# Autodesk Inventor assembly: HCMUTE-CDT23-PLXR_ASEMBLY
(part 2 of 2)
- Mate:182: HCMUTE-CDT23-MOTOR_DC24V-100RPM-XD42GA775:1 ↔ HCMUTE-CDT23-GA_DC:1
- Mate:183: HCMUTE-CDT23-MOTOR_DC24V-100RPM-XD42GA775:1 ↔ HCMUTE-CDT23-PULLY_S5M-15X15X8:1
- Mate:184 (5 mm): HCMUTE-CDT23-PULLY_S5M-15X15X8:1 ↔ HCMUTE-CDT23-GA_DC:1
- Mate:185: HCMUTE-CDT23-FRAME_ASEMBLY:1 ↔ HCMUTE-CDT23-GA_DC:1
- Mate:186 (59.9799 mm): HCMUTE-CDT23-FRAME_ASEMBLY:1 ↔ HCMUTE-CDT23-GA_DC:1
- Flush:25: HCMUTE-CDT23-PULLY_S5M-30X15X12:2 ↔ HCMUTE-CDT23-PULLY_S5M-15X15X8:1
- Mate:187: HCMUTE-CDT23-PULLY_S5M-15X15X8:1 ↔ 2309HCMUTE-CDT23-BELT_S5M-355X71X15:1
- Mate:188 (1 mm): HCMUTE-CDT23-PULLY_S5M-15X15X8:1 ↔ 2309HCMUTE-CDT23-BELT_S5M-355X71X15:1
- Mate:189: HCMUTE-CDT23-TRUC_DAN:1 ↔ 2309HCMUTE-CDT23-BELT_S5M-355X71X15:1
- Mate:190: HCMUTE-CDT23-FRAME_ASEMBLY:1 ↔ HCMUTE-CDT23-BAT_TRUC_DAN:2
- Mate:191: HCMUTE-CDT23-BAT_TRUC_DAN:2 ↔ HCMUTE-CDT23-GOI_DO_KFL003:2
- Mate:192: HCMUTE-CDT23-BAT_TRUC_DAN:2 ↔ ISO 4762 M6 x 25:3
- Mate:193: HCMUTE-CDT23-BAT_TRUC_DAN:2 ↔ ISO 4762 M6 x 25:4
- Mate:194: HCMUTE-CDT23-BAT_TRUC_DAN:1 ↔ ISO 4762 M6 x 12:1
- Mate:196: HCMUTE-CDT23-BAT_TRUC_DAN:1 ↔ ISO 4762 M6 x 12:2
- Mate:199: HCMUTE-CDT23-OP_GA-STEP-42:1 ↔ HCMUTE-CDT23-OP_NDH-2020X500:1
- Flush:26 (-9.75 mm): HCMUTE-CDT23-OP_GA-STEP-42:1 ↔ HCMUTE-CDT23-OP_NDH-2020X500:1
- Flush:27 (-40 mm): HCMUTE-CDT23-OP_GA-STEP-42:1 ↔ HCMUTE-CDT23-OP_NDH-2020X500:1
- Mate:200: HCMUTE-CDT23-OP_GA-STEP-42:1 ↔ HCMUTE-CDT23-OP_STEP-42:1
- Mate:201: HCMUTE-CDT23-OP_GA-STEP-42:1 ↔ HCMUTE-CDT23-OP_STEP-42:1
- Mate:202: HCMUTE-CDT23-OP_GA-CONLAN:1 ↔ HCMUTE-CDT23-OP_NDH-2020X500:1
- Flush:28 (-30 mm): HCMUTE-CDT23-OP_GA-CONLAN:1 ↔ HCMUTE-CDT23-OP_NDH-2020X500:1
- Mate:203 (3 mm): HCMUTE-CDT23-BTC_ASEMBLY:1 ↔ HCMUTE-CDT23-OP_NDH-2020X500:1
- Mate:206: HCMUTE-CDT23-FRAME_ASEMBLY:1 ↔ HCMUTE-CDT23-OP_TAMLOT:1
- Flush:30: HCMUTE-CDT23-FRAME_ASEMBLY:1 ↔ HCMUTE-CDT23-OP_TAMLOT:1
- Flush:31: HCMUTE-CDT23-OP_NDH-2020X500:1 ↔ HCMUTE-CDT23-OP_TAMLOT:1
- Mate:207: 301818 302828.1:1 ↔ HCMUTE-CDT23-OP_TAMLOT:1
- Mate:208: HCMUTE-CDT23-OP_NDH-2020X500:1 ↔ 301818 302828.1:1
- Flush:32 (6 mm): HCMUTE-CDT23-FRAME_ASEMBLY:1 ↔ 301818 302828.1:1
- Mate:209: HCMUTE-CDT23-OP_TAMLOT:1 ↔ 301818 302828.1:2
- Mate:210: HCMUTE-CDT23-OP_NDH-2020X500:1 ↔ 301818 302828.1:2
- Flush:33: 301818 302828.1:1 ↔ 301818 302828.1:2
- Mate:211: HCMUTE-CDT23-OP_TAMLOT:1 ↔ ISO 4762 M5 x 12:1
- Mate:212: 301818 302828.1:2 ↔ ISO 4762 M5 x 12:1
- Mate:213: HCMUTE-CDT23-OP_TAMLOT:1 ↔ ISO 4762 M5 x 12:2
- Mate:214: 301818 302828.1:1 ↔ ISO 4762 M5 x 12:2
- Flush:34 (-9.75 mm): HCMUTE-CDT23-OP_GA-CONLAN:1 ↔ HCMUTE-CDT23-OP_NDH-2020X500:1
- Flush:35 (-20 mm): HCMUTE-CDT23-FRAME_ASEMBLY:1 ↔ HCMUTE-CDT23-OP_NDH-2020X500:1
- Mate:215: HCMUTE-CDT23-OP_STEP-42:1 ↔ HCMUTE-CDT23-OP_PULLY-GT2-30X6X5:1
- Mate:216 (7 mm): HCMUTE-CDT23-OP_GA-STEP-42:1 ↔ HCMUTE-CDT23-OP_PULLY-GT2-30X6X5:1
- Mate:217: HCMUTE-CDT23-OP_GA-STEP-42:1 ↔ ISO 4762 M5 x 8:1
- Mate:218: HCMUTE-CDT23-OP_GA-STEP-42:1 ↔ ISO 4762 M5 x 8:1
- Mate:219: HCMUTE-CDT23-OP_GA-STEP-42:1 ↔ ISO 4762 M5 x 8:2
- Mate:220: HCMUTE-CDT23-OP_GA-STEP-42:1 ↔ ISO 4762 M5 x 8:2
- Mate:221: HCMUTE-CDT23-OP_GA-CONLAN:1 ↔ ISO 4762 M5 x 8:3
- Mate:222: HCMUTE-CDT23-OP_GA-CONLAN:1 ↔ ISO 4762 M5 x 8:3
- Mate:223: HCMUTE-CDT23-OP_GA-CONLAN:1 ↔ ISO 4762 M5 x 8:4
- Mate:224: HCMUTE-CDT23-OP_GA-CONLAN:1 ↔ ISO 4762 M5 x 8:4
- Mate:225: HCMUTE-CDT23-OP_GA-CONLAN:1 ↔ HCMUTE-CDT23-OP_RONG-ROC:1
- Mate:226: HCMUTE-CDT23-OP_GA-CONLAN:1 ↔ HCMUTE-CDT23-OP_RONG-ROC:1
- Mate:227: HCMUTE-CDT23-OP_V-WHEEL:1 ↔ HCMUTE-CDT23-OP_BASE-PLATE:1
- Mate:228: HCMUTE-CDT23-OP_V-WHEEL:1 ↔ HCMUTE-CDT23-OP_BASE-PLATE:1
- Mate:229: HCMUTE-CDT23-OP_BASE-PLATE:1 ↔ HCMUTE-CDT23-OP_V-WHEEL:3
- Mate:230: HCMUTE-CDT23-OP_BASE-PLATE:1 ↔ HCMUTE-CDT23-OP_V-WHEEL:3
- Mate:231: HCMUTE-CDT23-OP_BASE-PLATE:1 ↔ HCMUTE-CDT23-OP_V-WHEEL:4
- Mate:232: HCMUTE-CDT23-OP_BASE-PLATE:1 ↔ HCMUTE-CDT23-OP_V-WHEEL:4
- Mate:233: HCMUTE-CDT23-OP_BASE-PLATE:1 ↔ HCMUTE-CDT23-OP_V-WHEEL:5
- Mate:234: HCMUTE-CDT23-OP_BASE-PLATE:1 ↔ HCMUTE-CDT23-OP_V-WHEEL:5
- Angle:3 (0 deg): HCMUTE-CDT23-OP_BASE-PLATE:1
- Flush:37: HCMUTE-CDT23-OP_V-WHEEL:1
- Flush:38: HCMUTE-CDT23-OP_V-WHEEL:1
- Symmetry:1
- Flush:39: HCMUTE-CDT23-OP_NDH-2020X500:1
- Flush:40: HCMUTE-CDT23-OP_NDH-2020X500:1
- Symmetry:2
- Mate:235
- Mate:236: HCMUTE-CDT23-OP_GA-CONLAN:1 ↔ HCMUTE-CDT23-OP_BASE-PLATE:1
- Mate:273: HCMUTE-CDT23-OP_DVCAM:1 ↔ Assembly_HCMUTE-CDT23-CAMERA_C270Logitech c270 Assembly:1
- Mate:274: HCMUTE-CDT23-OP_DVCAM:1 ↔ Assembly_HCMUTE-CDT23-CAMERA_C270Logitech c270 Assembly:1
- Mate:275: HCMUTE-CDT23-OP_DVCAM:1 ↔ Assembly_HCMUTE-CDT23-CAMERA_C270Logitech c270 Assembly:1
- Mate:276: HCMUTE-CDT23-FRAME_ASEMBLY:1 ↔ HCMUTE-CDT23-KXL_CHAN-GA:1
- Flush:52 (-15 mm): HCMUTE-CDT23-FRAME_ASEMBLY:1 ↔ HCMUTE-CDT23-KXL_CHAN-GA:1
- Mate:277: HCMUTE-CDT23-FRAME_ASEMBLY:1 ↔ HCMUTE-CDT23-KXL_CHAN-GA:1
- Mate:278: HCMUTE-CDT23-KXL_CHAN-GA:1 ↔ ISO 4762 M6 x 10:10
- Mate:279: HCMUTE-CDT23-KXL_CHAN-GA:1 ↔ ISO 4762 M6 x 10:10
- Mate:280: HCMUTE-CDT23-KXL_CHAN-GA:1 ↔ ISO 4762 M6 x 10:9
- Mate:281: HCMUTE-CDT23-KXL_CHAN-GA:1 ↔ ISO 4762 M6 x 10:9
- Mate:282: HCMUTE-CDT23-FRAME_ASEMBLY:1 ↔ HCMUTE-CDT23-KXL_CHAN-GA:2
- Mate:283: HCMUTE-CDT23-FRAME_ASEMBLY:1 ↔ HCMUTE-CDT23-KXL_CHAN-GA:2
- Flush:53: HCMUTE-CDT23-KXL_CHAN-GA:1 ↔ HCMUTE-CDT23-KXL_CHAN-GA:2
- Mate:284 (6 mm): HCMUTE-CDT23-FRAME_ASEMBLY:1 ↔ HCMUTE-CDT23-KXL_CHAN-GA:3
- Mate:285: HCMUTE-CDT23-FRAME_ASEMBLY:1 ↔ HCMUTE-CDT23-KXL_CHAN-GA:3
- Flush:54: HCMUTE-CDT23-KXL_CHAN-GA:2 ↔ HCMUTE-CDT23-KXL_CHAN-GA:3
- Mate:286: HCMUTE-CDT23-KXL_CHAN-GA:1 ↔ HCMUTE-CDT23-KXL_A01:1
- Mate:287: HCMUTE-CDT23-KXL_CHAN-GA:1 ↔ HCMUTE-CDT23-KXL_A01:1
- Mate:288: HCMUTE-CDT23-KXL_A01:1 ↔ 2309HCMUTE-CDT23-KXL_GA-VUONG:1
- Flush:55: HCMUTE-CDT23-KXL_A01:1 ↔ 2309HCMUTE-CDT23-KXL_GA-VUONG:1
- Mate:289: HCMUTE-CDT23-KXL_A01:1 ↔ 2309HCMUTE-CDT23-KXL_GA-VUONG:1
- Mate:290: HCMUTE-CDT23-KXL_A01:1 ↔ 2309HCMUTE-CDT23-KXL_GA-VUONG:2
- Flush:56: 2309HCMUTE-CDT23-KXL_GA-VUONG:1 ↔ 2309HCMUTE-CDT23-KXL_GA-VUONG:2
- Mate:291: HCMUTE-CDT23-KXL_A01:1 ↔ 2309HCMUTE-CDT23-KXL_GA-VUONG:2
- Mate:292: HCMUTE-CDT23-KXL_A01:1 ↔ 2309HCMUTE-CDT23-KXL_GA-VUONG:3
- Mate:293: HCMUTE-CDT23-KXL_A01:1 ↔ 2309HCMUTE-CDT23-KXL_GA-VUONG:3
- Flush:57: HCMUTE-CDT23-KXL_A01:1 ↔ 2309HCMUTE-CDT23-KXL_GA-VUONG:3
- Mate:296: HCMUTE-CDT23-KXL_CHAN-GA:3 ↔ ISO 4032 M5:1
- Mate:309: 2309HCMUTE-CDT23-KXL_GA-VUONG:4 ↔ ISO 4032 M5:5
- Mate:310: ISO 4032 M5:5 ↔ ISO 4762 M5 x 12:8
- Mate:311: ISO 4032 M5:4 ↔ ISO 4762 M5 x 12:9
- Mate:312: ISO 4032 M5:4 ↔ 2309HCMUTE-CDT23-KXL_GA-VUONG:7
- Mate:313: HCMUTE-CDT23-KXL_A01:1 ↔ HCMUTE-CDT23-KXL_A03:1
- Mate:315: ISO 4762 M5 x 12:14 ↔ 2309HCMUTE-CDT23-KXL_GA-VUONG:7
- Mate:316: HCMUTE-CDT23-KXL_A03:1 ↔ ISO 4762 M5 x 12:14
- Mate:317: ISO 4032 M5:10 ↔ 2309HCMUTE-CDT23-KXL_GA-VUONG:7
- Mate:318: ISO 4032 M5:10 ↔ ISO 4762 M5 x 12:14
- Mate:319: HCMUTE-CDT23-KXL_A03:1 ↔ HCMUTE-CDT23-KXL_A02:2
- Flush:61: HCMUTE-CDT23-KXL_A03:1 ↔ HCMUTE-CDT23-KXL_A02:2
- Flush:62 (3 mm): HCMUTE-CDT23-KXL_A03:1 ↔ HCMUTE-CDT23-KXL_A02:2
- Mate:320: HCMUTE-CDT23-FRAME_ASEMBLY:1 ↔ HCMUTE-CDT23-KXL_CHAN-GA:4
- Flush:63 (-16 mm): HCMUTE-CDT23-FRAME_ASEMBLY:1 ↔ HCMUTE-CDT23-KXL_CHAN-GA:4
- Mate:321: HCMUTE-CDT23-FRAME_ASEMBLY:1 ↔ HCMUTE-CDT23-KXL_CHAN-GA:4
- Mate:322: HCMUTE-CDT23-FRAME_ASEMBLY:1 ↔ HCMUTE-CDT23-KXL_CHAN-GA:5
- Flush:64: HCMUTE-CDT23-KXL_CHAN-GA:4 ↔ HCMUTE-CDT23-KXL_CHAN-GA:5
- Flush:65: HCMUTE-CDT23-KXL_CHAN-GA:2 ↔ HCMUTE-CDT23-KXL_CHAN-GA:5
- Mate:323: HCMUTE-CDT23-FRAME_ASEMBLY:1 ↔ HCMUTE-CDT23-KXL_CHAN-GA:6
- Flush:66: HCMUTE-CDT23-KXL_CHAN-GA:4 ↔ HCMUTE-CDT23-KXL_CHAN-GA:6
- Flush:67: HCMUTE-CDT23-KXL_CHAN-GA:3 ↔ HCMUTE-CDT23-KXL_CHAN-GA:6
- Mate:324: HCMUTE-CDT23-KXL_CHAN-GA:6 ↔ HCMUTE-CDT23-KXL_A01:2
- Flush:68: HCMUTE-CDT23-KXL_CHAN-GA:6 ↔ HCMUTE-CDT23-KXL_A01:2
- Mate:325: HCMUTE-CDT23-KXL_CHAN-GA:6 ↔ HCMUTE-CDT23-KXL_A01:2
- Mate:326: HCMUTE-CDT23-KXL_CHAN-GA:5 ↔ HCMUTE-CDT23-KXL_A01:2
- Mate:327: HCMUTE-CDT23-KXL_CHAN-GA:6 ↔ ISO 4762 M6 x 10:15
- Mate:328: HCMUTE-CDT23-KXL_CHAN-GA:6 ↔ ISO 4762 M6 x 10:15
- Mate:329: HCMUTE-CDT23-KXL_CHAN-GA:6 ↔ ISO 4762 M6 x 10:16
- Mate:330: HCMUTE-CDT23-KXL_CHAN-GA:6 ↔ ISO 4762 M6 x 10:16
- Mate:331: HCMUTE-CDT23-KXL_A01:2 ↔ 2309HCMUTE-CDT23-KXL_GA-VUONG:10
- Mate:332: HCMUTE-CDT23-KXL_CHAN-GA:6 ↔ 2309HCMUTE-CDT23-KXL_GA-VUONG:10
- Mate:333: HCMUTE-CDT23-KXL_A02:2 ↔ 2309HCMUTE-CDT23-KXL_GA-VUONG:10
- Mate:334: HCMUTE-CDT23-KXL_A02:2 ↔ 2309HCMUTE-CDT23-KXL_GA-VUONG:11
- Mate:335: HCMUTE-CDT23-KXL_A02:2 ↔ 2309HCMUTE-CDT23-KXL_GA-VUONG:11
- Flush:69: HCMUTE-CDT23-KXL_A02:2 ↔ 2309HCMUTE-CDT23-KXL_GA-VUONG:11
- Mate:336: HCMUTE-CDT23-KXL_A02:2 ↔ 2309HCMUTE-CDT23-KXL_GA-VUONG:12
- Mate:337: HCMUTE-CDT23-KXL_A02:2 ↔ 2309HCMUTE-CDT23-KXL_GA-VUONG:12
- Mate:338: HCMUTE-CDT23-KXL_A03:1 ↔ 2309HCMUTE-CDT23-KXL_GA-VUONG:12
- Mate:339: 2309HCMUTE-CDT23-KXL_GA-VUONG:10 ↔ ISO 4762 M5 x 12:17
- Mate:340: HCMUTE-CDT23-KXL_CHAN-GA:6 ↔ ISO 4762 M5 x 12:17
- Mate:341: HCMUTE-CDT23-KXL_A02:2 ↔ ISO 4762 M5 x 12:20
- Mate:342: HCMUTE-CDT23-KXL_A02:2 ↔ ISO 4762 M5 x 12:20
- Mate:343: 2309HCMUTE-CDT23-KXL_GA-VUONG:10 ↔ ISO 4032 M5:15
- Mate:344: ISO 4032 M5:15 ↔ ISO 4762 M5 x 12:17
- Mate:345: 2309HCMUTE-CDT23-KXL_GA-VUONG:10 ↔ ISO 4032 M5:16
- Mate:346: ISO 4032 M5:16 ↔ ISO 4762 M5 x 12:20
- Mate:347: HCMUTE-CDT23-KXL_A02:2 ↔ ISO 4762 M5 x 12:18
- Mate:348: HCMUTE-CDT23-KXL_A02:2 ↔ ISO 4762 M5 x 12:18
- Mate:349: 2309HCMUTE-CDT23-KXL_GA-VUONG:11 ↔ ISO 4032 M5:14
- Mate:350: ISO 4762 M5 x 12:18 ↔ ISO 4032 M5:14
- Mate:351: HCMUTE-CDT23-KXL_A02:2 ↔ ISO 4762 M5 x 12:19
- Mate:352: HCMUTE-CDT23-KXL_A02:2 ↔ ISO 4762 M5 x 12:19
- Mate:353: ISO 4032 M5:13 ↔ ISO 4762 M5 x 12:19
- Mate:354: 2309HCMUTE-CDT23-KXL_GA-VUONG:12 ↔ ISO 4032 M5:13
- Mate:355: HCMUTE-CDT23-KXL_A03:1 ↔ ISO 4762 M5 x 12:27
- Mate:356: HCMUTE-CDT23-KXL_A03:1 ↔ ISO 4762 M5 x 12:27
- Mate:357: 2309HCMUTE-CDT23-KXL_GA-VUONG:12 ↔ ISO 4032 M5:23
- Mate:358: ISO 4762 M5 x 12:27 ↔ ISO 4032 M5:23
- Mate:360: HCMUTE-CDT23-KXL_A01:1 ↔ HCMUTE-CDT23-KXL_A04:1
- Mate:361: HCMUTE-CDT23-KXL_A04:1 ↔ ISO 4762 M5 x 12:32
- Mate:362: HCMUTE-CDT23-KXL_A04:1 ↔ ISO 4762 M5 x 12:32
- Mate:363: HCMUTE-CDT23-KXL_A04:1 ↔ ISO 4762 M5 x 12:33
- Mate:364: HCMUTE-CDT23-KXL_A04:1 ↔ ISO 4762 M5 x 12:33
- Mate:365: ISO 4032 M5:28 ↔ 2309HCMUTE-CDT23-KXL_GA-VUONG:4
- Mate:366: ISO 4032 M5:28 ↔ ISO 4762 M5 x 12:33
- Mate:367: 2309HCMUTE-CDT23-KXL_GA-VUONG:17 ↔ ISO 4032 M5:29
- Mate:368: ISO 4032 M5:29 ↔ ISO 4762 M5 x 12:32
- Mate:370: HCMUTE-CDT23-KXL_A03:1 ↔ HCMUTE-CDT23-KXL_A05:1
- Mate:371: HCMUTE-CDT23-KXL_A05:1 ↔ 2309HCMUTE-CDT23-KXL_GA-VUONG:19
- Flush:72: HCMUTE-CDT23-KXL_A05:1 ↔ 2309HCMUTE-CDT23-KXL_GA-VUONG:19
- Mate:372: HCMUTE-CDT23-KXL_A05:1 ↔ 2309HCMUTE-CDT23-KXL_GA-VUONG:19
- Mate:373: HCMUTE-CDT23-KXL_A04:1 ↔ 2309HCMUTE-CDT23-KXL_GA-VUONG:22
- Mate:374: HCMUTE-CDT23-KXL_A05:1 ↔ 2309HCMUTE-CDT23-KXL_GA-VUONG:22
- Mate:375: HCMUTE-CDT23-KXL_A05:1 ↔ 2309HCMUTE-CDT23-KXL_GA-VUONG:22
- Mate:376: 2309HCMUTE-CDT23-KXL_GA-VUONG:22 ↔ ISO 4032 M5:34
- Mate:377: 2309HCMUTE-CDT23-KXL_GA-VUONG:22 ↔ ISO 4032 M5:34
- Mate:378: 2309HCMUTE-CDT23-KXL_GA-VUONG:22 ↔ ISO 4032 M5:35
- Mate:379: 2309HCMUTE-CDT23-KXL_GA-VUONG:22 ↔ ISO 4032 M5:35
- Mate:380: HCMUTE-CDT23-KXL_A04:1 ↔ ISO 4762 M5 x 12:38
- Mate:381: HCMUTE-CDT23-KXL_A04:1 ↔ ISO 4762 M5 x 12:38
- Mate:382: HCMUTE-CDT23-KXL_A05:1 ↔ ISO 4762 M5 x 12:39
- Mate:383: HCMUTE-CDT23-KXL_A05:1 ↔ ISO 4762 M5 x 12:39
- Symmetry:3: HCMUTE-CDT23-KXL_A03:1 ↔ HCMUTE-CDT23-KXL_A04:1
- Mate:384: HCMUTE-CDT23-KXL_A05:1 ↔ Assembly_HCMUTE-CDT23-CAMERA_C270Logitech c270 Assembly:2
- Mate:385: HCMUTE-CDT23-KXL_A05:1 ↔ Assembly_HCMUTE-CDT23-CAMERA_C270Logitech c270 Assembly:2
- Mate:386: HCMUTE-CDT23-KXL_A05:1 ↔ Assembly_HCMUTE-CDT23-CAMERA_C270Logitech c270 Assembly:2
- Mate:399: HCMUTE-CDT23-FRAME_ASEMBLY:1 ↔ 2309HCMUTE-CDT23-BE_DO:1
- Flush:73: HCMUTE-CDT23-FRAME_ASEMBLY:1 ↔ 2309HCMUTE-CDT23-BE_DO:1
- Mate:400 (5 mm): HCMUTE-CDT23-BAT_TRUC_CANG_TAI:2 ↔ 2309HCMUTE-CDT23-BE_DO:1
- Tangent:1: Assembly_HCMUTE-CDT23-CYLINDER-AIRTAC_SC32X300:1 ↔ HCMUTE-CDT23-TAY_GAT:1
- Mate:401: Assembly_HCMUTE-CDT23-CYLINDER-AIRTAC_SC32X300:1 ↔ HCMUTE-CDT23-TAY_GAT:1
- Mate:402: HCMUTE-CDT23-FRAME_ASEMBLY:1 ↔ HCMUTE-CDT23-VND:1
- Flush:74: 2309HCMUTE-CDT23-BE_DO:1 ↔ HCMUTE-CDT23-VND:1
- Mate:403: Assembly_HCMUTE-CDT23-CYLINDER-AIRTAC_SC32X300:1 ↔ HCMUTE-CDT23-VND:1
- Mate:404: Assembly_HCMUTE-CDT23-CYLINDER-AIRTAC_SC32X300:1 ↔ HCMUTE-CDT23-VND:1
- Angle:6 (0 deg): Assembly_HCMUTE-CDT23-CYLINDER-AIRTAC_SC32X300:1 ↔ HCMUTE-CDT23-VND:1
- Mate:405: Assembly_HCMUTE-CDT23-CYLINDER-AIRTAC_SC32X300:1 ↔ 2309HCMUTE-CDT23-DO_GA:1
- Mate:406: Assembly_HCMUTE-CDT23-CYLINDER-AIRTAC_SC32X300:1 ↔ 2309HCMUTE-CDT23-DO_GA:1
- Mate:407: Assembly_HCMUTE-CDT23-CYLINDER-AIRTAC_SC32X300:1 ↔ 2309HCMUTE-CDT23-DO_GA:1
- Mate:408: HCMUTE-CDT23-VND:1 ↔ HCMUTE-CDT23-BAC_TRUOT:1
- Mate:409: HCMUTE-CDT23-VND:1 ↔ HCMUTE-CDT23-BAC_TRUOT:1
- Mate:410: HCMUTE-CDT23-VND:1 ↔ HCMUTE-CDT23-BAC_TRUOT:1
- Mate:411: HCMUTE-CDT23-BAC_TRUOT:1 ↔ HCMUTE-CDT23-TRUC_TRUOT:1
- Flush:76 (-10 mm): HCMUTE-CDT23-TAY_GAT:1 ↔ HCMUTE-CDT23-TRUC_TRUOT:1
- Mate:412: HCMUTE-CDT23-TAY_GAT:1 ↔ HCMUTE-CDT23-TRUC_TRUOT:1
- Flush:77: HCMUTE-CDT23-BAT_CANG_BANG_TAI:2 ↔ HCMUTE-CDT23-VND:1
- Mate:413: HCMUTE-CDT23-VND:1 ↔ Assembly_HCMUTE-CDT23-CB_E3F-DS30C4:1
- Mate:414: HCMUTE-CDT23-VND:1 ↔ Assembly_HCMUTE-CDT23-CB_E3F-DS30C4:1
- Angle:7 (0 deg): Assembly_HCMUTE-CDT23_BE-TRUOT:1
- Angle:8 (0 deg): Assembly_HCMUTE-CDT23_BE-TRUOT:1
- Mate:415: HCMUTE-CDT23-BAT_TRUC_CANG_TAI:1 ↔ Assembly_HCMUTE-CDT23_BE-TRUOT:1
- Mate:416: HCMUTE-CDT23-BAT_TRUC_CANG_TAI:1 ↔ Assembly_HCMUTE-CDT23_BE-TRUOT:1
- Mate:417: Assembly_HCMUTE-CDT23_BE-TRUOT:1 ↔ ISO 4762 M6 x 16:38
- Mate:418: Assembly_HCMUTE-CDT23_BE-TRUOT:1 ↔ ISO 4762 M6 x 16:38
- Mate:419: HCMUTE-CDT23-BAT_TRUC_CANG_TAI:1 ↔ Assembly_HCMUTE-CDT23_BE-TRUOT:1
- Mate:420: Assembly_HCMUTE-CDT23_BE-TRUOT:1 ↔ ISO 4762 M6 x 16:39
- Mate:421: Assembly_HCMUTE-CDT23_BE-TRUOT:1 ↔ ISO 4762 M6 x 16:39
- Mate:422 (20 mm): HCMUTE-CDT23-BAT_TRUC_CANG_TAI:1 ↔ HCMUTE-CDT23-TRUC_CANG:1
- Mate:423: HCMUTE-CDT23-BTC_ASEMBLY:1 ↔ 2309HCMUTE-CDT23-KXL_GA-VUONG:25
- Flush:78 (2 mm): HCMUTE-CDT23-BTC_ASEMBLY:1 ↔ 2309HCMUTE-CDT23-KXL_GA-VUONG:25
- Mate:424: HCMUTE-CDT23-BTC-VND:1 ↔ 2309HCMUTE-CDT23-KXL_GA-VUONG:25
- Mate:425: HCMUTE-CDT23-BTC_ASEMBLY:1 ↔ HCMUTE-CDT23-BTC-VND:1
- Mate:426: HCMUTE-CDT23-BTC_ASEMBLY:1 ↔ HCMUTE-CDT23-OP_NDH-2020X500:1
- Flush:80 (-22.75 mm): HCMUTE-CDT23-OP_NDH-2020X500:1 ↔ HCMUTE-CDT23-OP_BASE-PLATE:1
- Mate:427: HCMUTE-CDT23-OP_BASE-PLATE:1 ↔ HCMUTE-CDT23-OP_DVCAM:1
- Mate:428: HCMUTE-CDT23-OP_BASE-PLATE:1 ↔ HCMUTE-CDT23-OP_DVCAM:1
- Angle:9 (0 deg): HCMUTE-CDT23-OP_BASE-PLATE:1 ↔ HCMUTE-CDT23-OP_DVCAM:1
- Flush:81 (-9.75 mm): HCMUTE-CDT23-OP_GA-CONLAN3:1 ↔ HCMUTE-CDT23-OP_NDH-2020X5003:1
- Flush:82 (-30 mm): HCMUTE-CDT23-OP_GA-CONLAN3:1 ↔ HCMUTE-CDT23-OP_NDH-2020X5003:1
- Mate:429: HCMUTE-CDT23-OP_GA-CONLAN3:1 ↔ HCMUTE-CDT23-OP_NDH-2020X5003:1
- Flush:83 (-40 mm): HCMUTE-CDT23-OP_GA-STEP-423:1 ↔ HCMUTE-CDT23-OP_NDH-2020X5003:1
- Flush:84 (-9.75 mm): HCMUTE-CDT23-OP_GA-STEP-423:1 ↔ HCMUTE-CDT23-OP_NDH-2020X5003:1
- Mate:430: HCMUTE-CDT23-OP_GA-STEP-423:1 ↔ HCMUTE-CDT23-OP_NDH-2020X5003:1
- Mate:431: HCMUTE-CDT23-OP_GA-STEP-423:1 ↔ HCMUTE-CDT23-OP_STEP-423:1
- Mate:432: HCMUTE-CDT23-OP_GA-STEP-423:1 ↔ HCMUTE-CDT23-OP_STEP-423:1
- Mate:433: HCMUTE-CDT23-OP_NDH-2020X5003:1 ↔ 301818 302828.1:3
- Mate:434: 301818 302828.1:3 ↔ HCMUTE-CDT23-OP_TAMLOT3:1
- Flush:85: HCMUTE-CDT23-OP_NDH-2020X5003:1 ↔ HCMUTE-CDT23-OP_TAMLOT3:1
- Flush:86: 301818 302828.1:3 ↔ 301818 302828.1:4
- Mate:435: HCMUTE-CDT23-OP_NDH-2020X5003:1 ↔ 301818 302828.1:4
- Mate:436: HCMUTE-CDT23-OP_TAMLOT3:1 ↔ 301818 302828.1:4
- Mate:437: 301818 302828.1:4 ↔ ISO 4762 M5 x 12:50
- Mate:439: 301818 302828.1:3 ↔ ISO 4762 M5 x 12:51
- Mate:441 (7 mm): HCMUTE-CDT23-OP_GA-STEP-423:1 ↔ HCMUTE-CDT23-OP_PULLY-GT2-30X6X53:1
- Mate:442: HCMUTE-CDT23-OP_STEP-423:1 ↔ HCMUTE-CDT23-OP_PULLY-GT2-30X6X53:1
- Mate:443: HCMUTE-CDT23-OP_GA-STEP-423:1 ↔ ISO 4762 M5 x 8:5
- Mate:445: HCMUTE-CDT23-OP_GA-STEP-423:1 ↔ ISO 4762 M5 x 8:6
- Mate:447: HCMUTE-CDT23-OP_GA-CONLAN3:1 ↔ ISO 4762 M5 x 8:7
- Mate:449: HCMUTE-CDT23-OP_GA-CONLAN3:1 ↔ ISO 4762 M5 x 8:8
- Mate:451: HCMUTE-CDT23-OP_GA-CONLAN3:1 ↔ HCMUTE-CDT23-OP_RONG-ROC3:1
- Mate:452: HCMUTE-CDT23-OP_GA-CONLAN3:1 ↔ HCMUTE-CDT23-OP_RONG-ROC3:1
- Flush:87 (-22.75 mm): HCMUTE-CDT23-OP_NDH-2020X5003:1 ↔ HCMUTE-CDT23-OP_BASE-PLATE3:1
- Mate:453: HCMUTE-CDT23-OP_GA-CONLAN3:1 ↔ HCMUTE-CDT23-OP_BASE-PLATE3:1
- Angle:10 (0 deg): HCMUTE-CDT23-OP_BASE-PLATE3:1
- Mate:454: HCMUTE-CDT23-OP_V-WHEEL1:1 ↔ HCMUTE-CDT23-OP_BASE-PLATE3:1
- Mate:455: HCMUTE-CDT23-OP_V-WHEEL1:1 ↔ HCMUTE-CDT23-OP_BASE-PLATE3:1
- Mate:456: HCMUTE-CDT23-OP_BASE-PLATE3:1 ↔ HCMUTE-CDT23-OP_V-WHEEL1:2
- Mate:457: HCMUTE-CDT23-OP_BASE-PLATE3:1 ↔ HCMUTE-CDT23-OP_V-WHEEL1:2
- Mate:458: HCMUTE-CDT23-OP_BASE-PLATE3:1 ↔ HCMUTE-CDT23-OP_V-WHEEL1:3
- Mate:459: HCMUTE-CDT23-OP_BASE-PLATE3:1 ↔ HCMUTE-CDT23-OP_V-WHEEL1:3
- Mate:460: HCMUTE-CDT23-OP_BASE-PLATE3:1 ↔ HCMUTE-CDT23-OP_V-WHEEL1:4
- Mate:461: HCMUTE-CDT23-OP_BASE-PLATE3:1 ↔ HCMUTE-CDT23-OP_V-WHEEL1:4
- Flush:88: HCMUTE-CDT23-OP_V-WHEEL1:1
- Flush:89: HCMUTE-CDT23-OP_V-WHEEL1:1
- Flush:90: HCMUTE-CDT23-OP_NDH-2020X5003:1
- Flush:91: HCMUTE-CDT23-OP_NDH-2020X5003:1
- Flush:92: HCMUTE-CDT23-BTC_ASEMBLY:1 ↔ HCMUTE-CDT23-BTC-VND:1
- Mate:462: HCMUTE-CDT23-BTC_ASEMBLY:1 ↔ HCMUTE-CDT23-BTC-VND:2
- Flush:93: HCMUTE-CDT23-BTC_ASEMBLY:1 ↔ HCMUTE-CDT23-BTC-VND:2
- Flush:94: HCMUTE-CDT23-BTC-VND:1 ↔ HCMUTE-CDT23-BTC-VND:2
- Flush:95 (100 mm): HCMUTE-CDT23-BTC_ASEMBLY:1 ↔ 2309HCMUTE-CDT23-KXL_GA-VUONG:25
- Mate:463: 2309HCMUTE-CDT23-KXL_GA-VUONG:25 ↔ ISO 4762 M5 x 12:53
- Mate:464: 2309HCMUTE-CDT23-KXL_GA-VUONG:25 ↔ ISO 4762 M5 x 12:53
- Mate:465: 2309HCMUTE-CDT23-KXL_GA-VUONG:25 ↔ ISO 4762 M5 x 12:52
- Mate:466: 2309HCMUTE-CDT23-KXL_GA-VUONG:25 ↔ ISO 4762 M5 x 12:52
- Mate:467: ISO 4762 M5 x 12:53 ↔ ISO 4032 M5:46
- Mate:468: HCMUTE-CDT23-BTC-VND:1 ↔ ISO 4032 M5:46
- Mate:469: 2309HCMUTE-CDT23-KXL_GA-VUONG1:1 ↔ ISO 4762 M5 x 12:63
- Mate:471: 2309HCMUTE-CDT23-KXL_GA-VUONG1:1 ↔ ISO 4762 M5 x 12:62
- Mate:473: ISO 4762 M5 x 12:62 ↔ ISO 4032 M5:51
- Mate:474: HCMUTE-CDT23-KXL_A02:2 ↔ Assembly_HCMUTE-CDT23-CB_E3F-DS30C4:2
- Mate:475: HCMUTE-CDT23-KXL_A02:2 ↔ Assembly_HCMUTE-CDT23-CB_E3F-DS30C4:2
- Mate:476: 2309HCMUTE-CDT23-KXL_GA-VUONG:1 ↔ HCMUTE-CDT23-KXL_A06:1
- Mate:477: 2309HCMUTE-CDT23-KXL_GA-VUONG:1 ↔ HCMUTE-CDT23-KXL_A06:1
- Mate:478: 2309HCMUTE-CDT23-KXL_GA-VUONG:3 ↔ HCMUTE-CDT23-KXL_A06:1
- Mate:479: ISO 4032 M5:60 ↔ ISO 4762 M5 x 12:77
- Mate:480: ISO 4032 M5:61 ↔ ISO 4762 M5 x 12:76
- Mate:481: HCMUTE-CDT23-KXL_A05:1 ↔ ISO 4762 M4 x 16:3
- Mate:482: HCMUTE-CDT23-KXL_A05:1 ↔ ISO 4762 M4 x 16:2
- Mate:483: HCMUTE-CDT23-KXL_A05:1 ↔ ISO 4762 M4 x 16:1
- Mate:484: HCMUTE-CDT23-KXL_A05:1 ↔ ISO 4762 M4 x 16:4
- Mate:485: HCMUTE-CDT23-KXL_A05:1 ↔ ISO 4762 M4 x 16:4
- Mate:486: HCMUTE-CDT23-KXL_A05:1 ↔ ISO 4762 M4 x 16:1
- Mate:487: HCMUTE-CDT23-KXL_A05:1 ↔ ISO 4762 M4 x 16:2
- Mate:488: HCMUTE-CDT23-KXL_A05:1 ↔ ISO 4762 M4 x 16:3
- Mate:489: ISO 4762 M4 x 16:2 ↔ ISO 4032 M4:1
- Mate:490: ISO 4762 M4 x 16:1 ↔ ISO 4032 M4:2
- Mate:491: ISO 4762 M4 x 16:3 ↔ ISO 4032 M4:3
- Mate:492: ISO 4762 M4 x 16:4 ↔ ISO 4032 M4:4
- Mate:493: Assembly_HCMUTE-CDT23-CAMERA_C270Logitech c270 Assembly:2 ↔ ISO 4032 M4:3
- Mate:494: Assembly_HCMUTE-CDT23-CAMERA_C270Logitech c270 Assembly:2 ↔ ISO 4032 M4:1
- Mate:495: Assembly_HCMUTE-CDT23-CAMERA_C270Logitech c270 Assembly:2 ↔ ISO 4032 M4:4
- Mate:496: Assembly_HCMUTE-CDT23-CAMERA_C270Logitech c270 Assembly:2 ↔ ISO 4032 M4:2
- Mate:497: HCMUTE-CDT23-BTC_ASEMBLY:1 ↔ HCMUTE-CDT23-GOI_DO_KFL003:3
## Named parameters: d80_d73 = 0 mm, d81_d75 = 0 mm, d82_d76 = 0 mm, d83_d77 = 0 mm, d151_d112 = 0 mm, d152_d113 = 0 mm, d153_d114 = 0 mm, d154_d115 = 0 mm, d155_d121 = 0 mm, d156_d122 = 0 mm, d157_d123 = 0 mm, d158_d124 = 0 mm, d159_d110 = 0 mm, d160_d111 = 0 mm, d161_d125 = 0 mm, d162_d126 = 0 mm, d163_d127 = 0 mm, d164_d128 = 0 mm, d165_d129 = 0 mm, d166_d133 = 0 mm, d167_d134 = 0 mm, d168_d135 = -1.5 mm, d169_d149 = 0 mm, d170_d150 = 0 mm, d171_d136 = 0 mm, d172_d137 = 0 mm, d173_d138 = 0 mm, d174_d139 = 0 mm, d175_d140 = 0 mm, d176_d141 = 0 mm, d177_d142 = 0 mm, d178_d143 = 0 mm, d179_d144 = 0 mm, d180_d145 = 0 mm, d181_d146 = 0 mm, d182_d147 = 0 mm, d183_d148 = 0 mm
